# Autodesk Inventor assembly: 4834267 DPDM-Q-16-50-PA---(0)
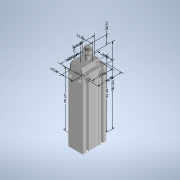
[picture p0: Inventor's stored thumbnail of the model, 180x180]
Saved by Autodesk Inventor 2021 (Build 250183000, 183)
## iProperties
Category: PARTsolutions
Company: FESTO
Created: 2026-04-25
Part Number: 4834267 DPDM-Q-16-50-PA---(0)
Catalog Web Link: www.3dfindit.com
Description: DPDM-compact cylinder
Vendor: FESTO
Document SubType Name: Assembly
Designer: psAdmin
Manufacturer: FESTO
Mass: 142.5 g
Surface Area: 234.053 cm^2
Volume: 44.6453 cm^3
Density: 3.19182 g/cm^3
Title: 4834267 DPDM-Q-16-50-PA
Author: Cadenas PARTsolutions
Comments: compact cylinder
PSOL_IDENT_0: {ATYP=ASSISTANT},{DATA=script=$CADENAS_DATA/23d-libs/festo/webfesto.vbb&M_FAMILY=DPDM&M_GROUP=01&M_P
PSOL_IDENT_1: ARTNO=4834267&IDCODE1=DPDM-Q-16-50-PA&IDCODE2=&customer_number_cns=&MATES=1&LOD=HI&LOCKERP=0&SINGLEP
PSOL_IDENT_2: ART=1}
NB: 4834267 DPDM-Q-16-50-PA---(0)
NN: DPDM
NT: compact cylinder
NBSYN: $TNR. $TYP.$VERNB.-$KOL.-$HUB.$FUNNB.$KOTNB.-$DAEM.$POS.$TEMNB.$BWENB.---($HUBST.)
LINA: 4834267 DPDM-Q-16-50-PA
CATALOG: Festo
TNR: 4834267
TYP: DPDM
VER: Q
KOL: 16
HUB: 50
HUBST: 0
FUN: -
KOT: -
DAEM: P
POS: A
TEM: -
BWE: -
AM: 12
KK: M6
WH: 5
MM: 6
SW: 5
LS: 3
ZJ: 45
L2: 40
EE: M5
ET: 4.5
BG: 6
RT: M4
H2: 19
E: 20
UO: 32
TO: 27
H3: 13
LX: 7
PL: 24.1
PR: 11
U1: 0
D5: 4.3
D6: 7.5
T1: 6
B3: 15
H4: 15.5
H5: 24
L4: 52
L5: 12
L6: 3
ZM: 50
L8: 57
D8: 2.3
W22: 3
H7: 10
H8: 3.2
CNSMASSEXACT: 0.1425
GTIN: 4052568293215
SUPPLIER: FESTO
ARTICLENO: 4834267 DPDM-Q-16-50-PA---(0)
BOMINFO: 4834267 DPDM-Q-16-50-PA
CREATOR: CADENAS GmbH
## Documents named in this file (6)
- e:\temp\worker_COMMON_269\temp\tmp_5480_0_lT3Hw\format_0\4834267 DPDM-Q-16-50-PA---(0).iam
- e:\temp\worker_COMMON_269\temp\tmp_5480_0_lT3Hw\format_0\4186566 DPDM-Q-50---(h).ipt
- e:\temp\worker_COMMON_269\temp\tmp_5480_0_lT3Hw\format_0\4186566 DPDM-Q-50---(r).ipt
- e:\temp\worker_COMMON_269\temp\tmp_5480_0_lT3Hw\format_0\ISO 4035 M6(F).ipt
- e:\temp\worker_COMMON_269\temp\tmp_5480_0_lT3Hw\format_0\4186566 DPDM 16-50---(p).ipt
- e:\temp\worker_COMMON_269\temp\tmp_5480_0_lT3Hw\format_0\ISO-4762 M3x10.ipt
## Components (5 placed, 5 different names)
1. 4186566 DPDM-Q-50---(h):1 — CP_ROD1_XY@1 <-> CP1_XY@2, CP_ROD1_Z@1 <-> CP1_Z@2, CP_ROD1_YZ@1 <-> CP1_YZ@2
2. 4186566 DPDM-Q-50---(r):1 — CP_ROD1_XY@1 <-> CP1_XY@2, CP_ROD1_Z@1 <-> CP1_Z@2, CP_ROD1_YZ@1 <-> CP1_YZ@2, NUT_CP_6_10_2_XY@2 <-> IP2_XY@3, NUT_CP_6_10_2_Z@2 <-> IP2_Z@3, NUT_CP_6_10_2_YZ@2 <-> IP2_YZ@3, CP_PL_XY@2 <-> CP_PLATE_XY@4, CP_PL_Z@2 <-> CP_PLATE_Z@4, CP_PL_YZ@2 <-> CP_PLATE_YZ@4
3. ISO 4035 M6(F):1 — NUT_CP_6_10_2_XY@2 <-> IP2_XY@3, NUT_CP_6_10_2_Z@2 <-> IP2_Z@3, NUT_CP_6_10_2_YZ@2 <-> IP2_YZ@3
4. 4186566 DPDM 16-50---(p):1 — CP_PL_XY@2 <-> CP_PLATE_XY@4, CP_PL_Z@2 <-> CP_PLATE_Z@4, CP_PL_YZ@2 <-> CP_PLATE_YZ@4, CP_SCREW_XY@4 <-> ANBAU_XY@5, CP_SCREW_Z@4 <-> ANBAU_Z@5, CP_SCREW_YZ@4 <-> ANBAU_YZ@5
5. ISO-4762 M3x10:1 — CP_SCREW_XY@4 <-> ANBAU_XY@5, CP_SCREW_Z@4 <-> ANBAU_Z@5, CP_SCREW_YZ@4 <-> ANBAU_YZ@5
## Relationships (12: Mate 5, Angle 4, Flush 3)
- CP_ROD1_XY@1 <-> CP1_XY@2 [Mate]: 4186566 DPDM-Q-50---(h):1 ↔ 4186566 DPDM-Q-50---(r):1
- CP_ROD1_Z@1 <-> CP1_Z@2 [Mate]: 4186566 DPDM-Q-50---(h):1 ↔ 4186566 DPDM-Q-50---(r):1
- CP_ROD1_YZ@1 <-> CP1_YZ@2 [Angle] (0 deg): 4186566 DPDM-Q-50---(h):1 ↔ 4186566 DPDM-Q-50---(r):1
- NUT_CP_6_10_2_XY@2 <-> IP2_XY@3 [Flush]: 4186566 DPDM-Q-50---(r):1 ↔ ISO 4035 M6(F):1
- NUT_CP_6_10_2_Z@2 <-> IP2_Z@3 [Mate]: 4186566 DPDM-Q-50---(r):1 ↔ ISO 4035 M6(F):1
- NUT_CP_6_10_2_YZ@2 <-> IP2_YZ@3 [Angle] (0 deg): 4186566 DPDM-Q-50---(r):1 ↔ ISO 4035 M6(F):1
- CP_PL_XY@2 <-> CP_PLATE_XY@4 [Flush]: 4186566 DPDM-Q-50---(r):1 ↔ 4186566 DPDM 16-50---(p):1
- CP_PL_Z@2 <-> CP_PLATE_Z@4 [Mate]: 4186566 DPDM-Q-50---(r):1 ↔ 4186566 DPDM 16-50---(p):1
- CP_PL_YZ@2 <-> CP_PLATE_YZ@4 [Angle] (0 deg): 4186566 DPDM-Q-50---(r):1 ↔ 4186566 DPDM 16-50---(p):1
- CP_SCREW_XY@4 <-> ANBAU_XY@5 [Flush]: 4186566 DPDM 16-50---(p):1 ↔ ISO-4762 M3x10:1
- CP_SCREW_Z@4 <-> ANBAU_Z@5 [Mate]: 4186566 DPDM 16-50---(p):1 ↔ ISO-4762 M3x10:1
- CP_SCREW_YZ@4 <-> ANBAU_YZ@5 [Angle] (0 deg): 4186566 DPDM 16-50---(p):1 ↔ ISO-4762 M3x10:1
